# Autodesk Inventor assembly: end door assembly (9).ipt
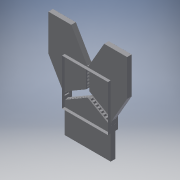
[picture p0: Inventor's stored thumbnail of the model, 180x180]
Saved by Autodesk Inventor 2017 (Build 210142000, 142)
## iProperties
Created: 2018-03-30
Part Number: end door assembly (9).ipt
Document SubType Name: Assembly
Designer: Braxton
Author: Braxton
## Documents named in this file (5)
- D:\School\Game develpment\geoscape\done\single wall\doors (one wall)\9 foot door (one wall)\end door assembly (one wall) (9).ipt.iam
- D:\School\Game develpment\geoscape\done\single wall\doors (one wall)\9 foot door (one wall)\bottom door (one wall) (9).ipt
- D:\School\Game develpment\geoscape\done\single wall\doors (one wall)\9 foot door (one wall)\end door frame (one wall) (9).ipt
- D:\School\Game develpment\geoscape\done\single wall\doors (one wall)\9 foot door (one wall)\top left door (one wall) (9).ipt
- D:\School\Game develpment\geoscape\done\single wall\doors (one wall)\9 foot door (one wall)\top right door (one wall) (9).ipt
## Components (4 placed, 4 different names)
1. end door frame (one wall) (9):1 — Mate:2, Mate:6, Mate:7, Mate:8, Mate:9, Mate:10
2. bottom door (one wall) (9):1 — Mate:2, Flush:2
3. top left door (one wall) (9):1 — Mate:6, Mate:9, Flush:1, Mate:10, Flush:2, Flush:3
4. top right door (one wall) (9):1 — Mate:7, Mate:8, Flush:1, Flush:3
## Relationships (9: Mate 6, Flush 3)
- Mate:2: end door frame (one wall) (9):1 ↔ bottom door (one wall) (9):1
- Mate:6: end door frame (one wall) (9):1 ↔ top left door (one wall) (9):1
- Mate:7: end door frame (one wall) (9):1 ↔ top right door (one wall) (9):1
- Mate:8: end door frame (one wall) (9):1 ↔ top right door (one wall) (9):1
- Mate:9: end door frame (one wall) (9):1 ↔ top left door (one wall) (9):1
- Flush:1: top left door (one wall) (9):1 ↔ top right door (one wall) (9):1
- Mate:10: end door frame (one wall) (9):1 ↔ top left door (one wall) (9):1
- Flush:2: bottom door (one wall) (9):1 ↔ top left door (one wall) (9):1
- Flush:3: top left door (one wall) (9):1 ↔ top right door (one wall) (9):1
